# Autodesk Inventor assembly: Gesamt
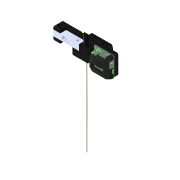
[picture p0: Inventor's stored thumbnail of the model, 180x180]
Saved by Autodesk Inventor 2022 (Build 260153000, 153)
## iProperties
Created: 2021-05-08
Part Number: Gesamt
Document SubType Name: Assembly
Designer: Sven
Author: Sven
## Documents named in this file (8)
- C:\Users\Sven\Documents\MesstechnikPraktikumV6\hardware\cad\Gesamt.iam
- C:\Users\Sven\Documents\MesstechnikPraktikumV6\hardware\cad\micro load cell CZL635.ipt
- C:\Users\Sven\Documents\MesstechnikPraktikumV6\hardware\cad\Flansch_Simple.ipt
- C:\Users\Sven\Documents\MesstechnikPraktikumV6\hardware\cad\Abdeckung_Sensorplatine.ipt
- C:\Users\Sven\Documents\MesstechnikPraktikumV6\hardware\cad\NadelHalterLose.ipt
- C:\Users\Sven\Documents\MesstechnikPraktikumV6\hardware\cad\NadelhalterSchraub.ipt
- C:\Users\Sven\Documents\MesstechnikPraktikumV6\hardware\cad\Nadel.ipt
- C:\Users\Sven\Documents\MesstechnikPraktikumV6\hardware\cad\LowPolyMessplatine.ipt
## Components (7 placed, 7 different names)
1. Flansch_Simple:1 — Passend:12, Passend:13, Passend:14, Fluchtend:3, Fluchtend:4, Passend:19
2. micro load cell CZL635:1 — Passend:8, Passend:9, Passend:10
3. Abdeckung_Sensorplatine:1
4. NadelHalterLose:1 — Passend:11, Fluchtend:1, Fluchtend:2, Passend:14, Passend:17, Passend:18, Winkel:1
5. NadelhalterSchraub:1 — Passend:8, Passend:9, Passend:10, Passend:11, Fluchtend:1, Fluchtend:2, Passend:12, Passend:13
6. Nadel:1 — Passend:17, Passend:18, Winkel:1
7. LowPolyMessplatine:1 — Fluchtend:3, Fluchtend:4, Passend:19
## Relationships (15: Mate 10, Flush 4, Angle 1)
- Passend:8 [Mate]: micro load cell CZL635:1 ↔ NadelhalterSchraub:1
- Passend:9 [Mate]: micro load cell CZL635:1 ↔ NadelhalterSchraub:1
- Passend:10 [Mate]: micro load cell CZL635:1 ↔ NadelhalterSchraub:1
- Passend:11 [Mate]: NadelHalterLose:1 ↔ NadelhalterSchraub:1
- Fluchtend:1 [Flush]: NadelHalterLose:1 ↔ NadelhalterSchraub:1
- Fluchtend:2 [Flush]: NadelHalterLose:1 ↔ NadelhalterSchraub:1
- Passend:12 [Mate] (-20 mm): Flansch_Simple:1 ↔ NadelhalterSchraub:1
- Passend:13 [Mate] (5 mm): Flansch_Simple:1 ↔ NadelhalterSchraub:1
- Passend:14 [Mate] (1.25 mm): Flansch_Simple:1 ↔ NadelHalterLose:1
- Passend:17 [Mate]: NadelHalterLose:1 ↔ Nadel:1
- Passend:18 [Mate]: NadelHalterLose:1 ↔ Nadel:1
- Winkel:1 [Angle] (0 deg): NadelHalterLose:1 ↔ Nadel:1
- Fluchtend:3 [Flush]: Flansch_Simple:1 ↔ LowPolyMessplatine:1
- Fluchtend:4 [Flush]: Flansch_Simple:1 ↔ LowPolyMessplatine:1
- Passend:19 [Mate]: Flansch_Simple:1 ↔ LowPolyMessplatine:1
